# Autodesk Inventor assembly: recovery_asm
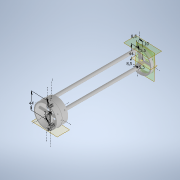
[picture p0: Inventor's stored thumbnail of the model, 180x180]
Saved by Autodesk Inventor 2020 (Build 240168000, 168)
## iProperties
Created: 2022-06-15
Part Number: recovery_asm
Document SubType Name: Assembly
Designer: sp
Author: sp
## Documents named in this file (4)
- C:\Users\sp\Desktop\neu_Rocket\recovery_asm.iam
- C:\Users\sp\Desktop\neu_Rocket\Verbindungsring_bottom.ipt
- C:\Users\sp\Desktop\neu_Rocket\stange.ipt
- C:\Users\sp\Desktop\neu_Rocket\Verbindungsring_top.ipt
## Components (4 placed, 3 different names)
1. Verbindungsring_bottom:1 — Einfügen:2, Einfügen:3
2. stange:1 — Einfügen:2, Einfügen:5
3. Verbindungsring_top:1 — Einfügen:4, Einfügen:5
4. stange:2 — Einfügen:3, Einfügen:4
## Relationships (4: Insert 4)
- Einfügen:2 [Insert]: Verbindungsring_bottom:1 ↔ stange:1
- Einfügen:3 [Insert]: Verbindungsring_bottom:1 ↔ stange:2
- Einfügen:4 [Insert]: Verbindungsring_top:1 ↔ stange:2
- Einfügen:5 [Insert]: stange:1 ↔ Verbindungsring_top:1
